# Autodesk Inventor assembly: cellSTORM_v5_microsocpe_alliedvision
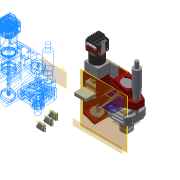
[picture p0: Inventor's stored thumbnail of the model, 180x180]
Saved by Autodesk Inventor 2019.4 (Build 234330000, 330)
## iProperties
Created: 2020-04-25
Part Number: cellSTORM_v5_microsocpe_alliedvision
Document SubType Name: Assembly
Designer: diederichbenedict
Author: diederichbenedict
## Documents named in this file (13)
- C:\Users\diederichbenedict\Dropbox\Dokumente\Promotion\PROJECTS\STORMoChip\GITHUB\CAD\Nanoscopy-on-the-cheap\Workspace\cellSTORM_v5_microsocpe_alliedvision.iam
- C:\Users\diederichbenedict\Dropbox\Dokumente\Promotion\PROJECTS\STORMoChip\GITHUB\CAD\Nanoscopy-on-the-cheap\Workspace\10_Filteslide_25mm.ipt
- C:\Users\diederichbenedict\Dropbox\Dokumente\Promotion\PROJECTS\STORMoChip\GITHUB\CAD\Nanoscopy-on-the-cheap\Workspace\cellSTORM_lightpath.ipt
- C:\Users\diederichbenedict\Dropbox\Dokumente\Promotion\PROJECTS\STORMoChip\GITHUB\CAD\Nanoscopy-on-the-cheap\Workspace\PF10-03-P01-Step.ipt
- C:\Users\diederichbenedict\Dropbox\Dokumente\Promotion\PROJECTS\STORMoChip\GITHUB\CAD\Nanoscopy-on-the-cheap\Workspace\cellSTORM_v5_opticalstage.ipt
- C:\Users\diederichbenedict\Dropbox\Dokumente\Promotion\PROJECTS\STORMoChip\GITHUB\CAD\Nanoscopy-on-the-cheap\Workspace\00_Micrometer.ipt
- C:\Users\diederichbenedict\Dropbox\Dokumente\Promotion\PROJECTS\STORMoChip\GITHUB\CAD\Nanoscopy-on-the-cheap\Workspace\Assembly_Z_stage.iam
- C:\Users\diederichbenedict\Dropbox\Dokumente\Promotion\PROJECTS\STORMoChip\GITHUB\CAD\Nanoscopy-on-the-cheap\Workspace\00_Alvium_Step_USB90_S-Mount_ClosedHousing_2019-Mar-28.ipt
- C:\Users\diederichbenedict\Dropbox\Dokumente\Promotion\PROJECTS\STORMoChip\GITHUB\CAD\Nanoscopy-on-the-cheap\Workspace\00_SM1L15-Step.ipt
- C:\Users\diederichbenedict\Dropbox\Dokumente\Promotion\PROJECTS\STORMoChip\GITHUB\CAD\Nanoscopy-on-the-cheap\Workspace\cellSTORM_ThorlabsTubeAdapter.ipt
- C:\Users\diederichbenedict\Dropbox\Dokumente\Promotion\PROJECTS\STORMoChip\GITHUB\CAD\Nanoscopy-on-the-cheap\Workspace\cellSTORM_Lensmount.ipt
- C:\Users\diederichbenedict\Dropbox\Dokumente\Promotion\PROJECTS\STORMoChip\GITHUB\CAD\Nanoscopy-on-the-cheap\Workspace\00_z-slider_chinese_OPPO.ipt
- C:\Users\diederichbenedict\Dropbox\Dokumente\Promotion\PROJECTS\STORMoChip\GITHUB\CAD\Nanoscopy-on-the-cheap\Workspace\00_Microscope_Objective.ipt
## Components (15 placed, 12 different names)
1. 10_Filteslide_25mm:1
2. PF10-03-P01-Step:1
3. PF10-03-P01-Step:2
4. cellSTORM_v5_opticalstage:1 — Insert:6, Flush:1, Flush:2, Insert:8, Mate:2, Angle:1
5. cellSTORM_lightpath:1 — Mate:1, Insert:10
6. 00_z-slider_chinese_OPPO:3
7. 00_z-slider_chinese_OPPO:2
8. 00_z-slider_chinese_OPPO:1
9. 00_Micrometer:1 — Insert:6
10. cellSTORM_ThorlabsTubeAdapter:1 — Flush:1, Flush:2
11. 00_Alvium_Step_USB90_S-Mount_ClosedHousing_2019-Mar-28:1 — Insert:8, Insert:9
12. 00_SM1L15-Step:1 — Insert:9
13. cellSTORM_Lensmount:1 — Mate:1, Mate:2, Angle:1
14. Assembly_Z_stage:1 [sub-assembly]
15. 00_Microscope_Objective:1 — Insert:10
## Relationships (12: Insert 7, Flush 2, Mate 2, Angle 1)
- [Insert]: PF10-03-P01-Step:1 ↔ cellSTORM_lightpath:1
- [Insert]: PF10-03-P01-Step:2 ↔ cellSTORM_lightpath:1
- [Insert] (40 mm): 10_Filteslide_25mm:1 ↔ cellSTORM_lightpath:1
- Insert:6: cellSTORM_v5_opticalstage:1 ↔ 00_Micrometer:1
- Flush:1: cellSTORM_v5_opticalstage:1 ↔ cellSTORM_ThorlabsTubeAdapter:1
- Flush:2: cellSTORM_v5_opticalstage:1 ↔ cellSTORM_ThorlabsTubeAdapter:1
- Insert:8 (-42 mm): cellSTORM_v5_opticalstage:1 ↔ 00_Alvium_Step_USB90_S-Mount_ClosedHousing_2019-Mar-28:1
- Insert:9: 00_Alvium_Step_USB90_S-Mount_ClosedHousing_2019-Mar-28:1 ↔ 00_SM1L15-Step:1
- Mate:1: cellSTORM_lightpath:1 ↔ cellSTORM_Lensmount:1
- Mate:2: cellSTORM_v5_opticalstage:1 ↔ cellSTORM_Lensmount:1
- Angle:1 (0 deg): cellSTORM_v5_opticalstage:1 ↔ cellSTORM_Lensmount:1
- Insert:10 (30 mm): cellSTORM_lightpath:1 ↔ 00_Microscope_Objective:1
